# Autodesk Inventor assembly: Hand Assembly V1
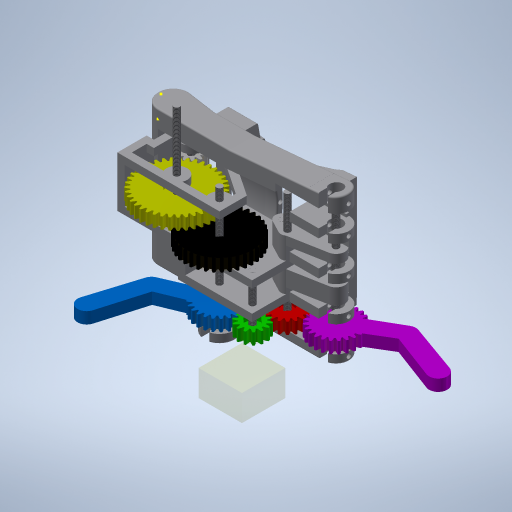
[picture p0: Inventor's stored thumbnail of the model, 512x512]
Saved by Autodesk Inventor 2023 (Build 270158000, 158)
## iProperties
Created: 2016-09-27
Part Number: Hand Assembly V1
Document SubType Name: Assembly
Designer: cmcdona
Author: cmcdona
## Documents named in this file (22)
- C:\Users\manny\OneDrive\Desktop\1C03 Stuff\Hand Assembly\Hand Assembly V1.iam
- C:\Users\manny\OneDrive\Desktop\1C03 Stuff\Hand Assembly\Hand - Frame.ipt
- C:\Users\manny\OneDrive\Desktop\1C03 Stuff\Hand Assembly\Hand - Digit 4.ipt
- C:\Users\manny\OneDrive\Desktop\1C03 Stuff\Hand Assembly\Hand - Digit 0-1.ipt
- C:\Users\manny\OneDrive\Desktop\1C03 Stuff\Hand Assembly\Hand - Distal Bridge.ipt
- C:\Users\manny\OneDrive\Desktop\1C03 Stuff\Hand Assembly\Hand - Digit 2-3.ipt
- C:\Users\manny\OneDrive\Desktop\1C03 Stuff\Hand Assembly\Hand - Proximal Bridge.ipt
- C:\Users\manny\OneDrive\Desktop\1C03 Stuff\Hand Assembly\Hand - Functional Workspace.ipt
- C:\Users\manny\OneDrive\Desktop\1C03 Stuff\Hand Assembly\Input Motor.ipt
- C:\Users\manny\OneDrive\Desktop\1C03 Stuff\Hand Assembly\Spur Gear11.ipt
- C:\Users\manny\OneDrive\Desktop\1C03 Stuff\Hand Assembly\Spur Gear22.ipt
- C:\Users\manny\OneDrive\Desktop\1C03 Stuff\Hand Assembly\temp back plate.ipt
- C:\Users\manny\OneDrive\Desktop\1C03 Stuff\Hand Assembly\Spur Gear12.ipt
- C:\Users\manny\OneDrive\Desktop\1C03 Stuff\Hand Assembly\Spur Gear23.ipt
- C:\Users\manny\OneDrive\Desktop\1C03 Stuff\Hand Assembly\Spur Gear21.ipt
- C:\Users\manny\OneDrive\Desktop\1C03 Stuff\Hand Assembly\FrameAssembly(Printing).iam
- C:\Users\manny\OneDrive\Desktop\1C03 Stuff\Hand Assembly\Spur Gear6.ipt
- C:\Users\manny\OneDrive\Desktop\1C03 Stuff\Hand Assembly\Spur Gear7.ipt
- C:\Users\manny\OneDrive\Desktop\1C03 Stuff\Hand Assembly\Threaded Rod.ipt
- C:\Users\manny\OneDrive\Desktop\1C03 Stuff\Hand Assembly\Threaded Rod 30mm.ipt
- C:\Users\manny\OneDrive\Desktop\1C03 Stuff\Hand Assembly\Threaded Rod38 mm.ipt
- C:\Users\manny\OneDrive\Desktop\1C03 Stuff\Hand Assembly\Threaded Rod 46mm.ipt
## Components (27 placed, 16 different names)
1. Hand - Frame:1 — Flush:1, Flush:2, Mate:1, Mate:2, Flush:3, Mate:3, Mate:16, Mate:17, Mate:18, Mate:33, Mate:34, Mate:53, Mate:66
2. Hand - Digit 4:1 — Flush:1, Flush:2, Mate:1, Mate:4, Mate:5
3. Hand - Digit 0-1:1 — Mate:2, Flush:3, Mate:3, Mate:6, Mate:19, Mate:20, Mate:21, Mate:31, Mate:58, Mate:59, Mate:63, Flush:21
4. Hand - Distal Bridge:1 — Mate:4, Mate:5, Mate:6, Mate:7, Mate:8, Mate:9, Mate:10, Mate:11, Mate:12, Mate:13, Mate:14, Mate:15
5. Hand - Digit 2-3:1 — Mate:7, Mate:8, Mate:9
6. Hand - Digit 2-3:2 — Mate:10, Mate:11, Mate:12
7. Hand - Digit 2-3:3 — Mate:13, Mate:14, Mate:15
8. Hand - Proximal Bridge:1 — Mate:16, Mate:17, Mate:18
9. Hand - Functional Workspace:1 — Mate:19, Mate:20, Mate:21
10. Input Motor:1 — Mate:24, Mate:25, Mate:32, Mate:33, Mate:34, Mate:53, Mate:54, Mate:65
11. Spur Gear1:1 — Mate:24, Flush:11, Mate:54, Tangent:3, Rotation:4
12. Spur Gear2:1 — Mate:27, Flush:11, Mate:64, Tangent:3, Mate:71, Mate:72, Rotation:4
13. Spur Gear1:2 — Mate:27, Mate:64, Flush:20, Tangent:2, Mate:71, Rotation:5
14. Spur Gear2:2 — Mate:31, Flush:20, Tangent:2, Mate:70, Rotation:5
15. Spur Gear2:3 — Mate:58, Mate:63, Flush:22, Rotation:1, Mate:70, Flush:27, Mate:76
16. Spur Gear2:4 — Mate:59, Mate:69, Rotation:3, Flush:24, Mate:73
17. Spur Gear1:3 — Mate:67, Flush:22, Flush:23, Rotation:1, Rotation:2, Mate:79, Flush:30
18. Spur Gear2:5 — Mate:68, Flush:23, Rotation:2, Rotation:3, Flush:25, Mate:74
19. FrameAssembly(Printing):1 [sub-assembly] — Mate:65, Flush:21, Mate:66, Mate:67, Mate:68, Mate:69, Mate:72, Flush:28, Mate:77, Flush:29, Mate:78, Mate:80, Flush:31
20. temp back plate:1 — Mate:25, Mate:32
21. Threaded Rod:1 — Flush:24, Mate:73
22. Threaded Rod:2 — Flush:25, Mate:74
23. Threaded Rod:4 — Flush:27, Mate:76
24. Threaded Rod:5 — Flush:28, Mate:77
25. Threaded Rod 30mm:1 — Flush:29, Mate:78
26. Threaded Rod38 mm:1 — Mate:79, Flush:30
27. Threaded Rod 46mm:1 — Mate:80, Flush:31
## Relationships (71: Mate 49, Flush 15, RelateRotation 5, Tangent 2)
- Flush:1: Hand - Frame:1 ↔ Hand - Digit 4:1
- Flush:2: Hand - Frame:1 ↔ Hand - Digit 4:1
- Mate:1: Hand - Frame:1 ↔ Hand - Digit 4:1
- Mate:2: Hand - Frame:1 ↔ Hand - Digit 0-1:1
- Flush:3: Hand - Frame:1 ↔ Hand - Digit 0-1:1
- Mate:3: Hand - Frame:1 ↔ Hand - Digit 0-1:1
- Mate:4: Hand - Digit 4:1 ↔ Hand - Distal Bridge:1
- Mate:5: Hand - Digit 4:1 ↔ Hand - Distal Bridge:1
- Mate:6: Hand - Digit 0-1:1 ↔ Hand - Distal Bridge:1
- Mate:7: Hand - Distal Bridge:1 ↔ Hand - Digit 2-3:1
- Mate:8: Hand - Distal Bridge:1 ↔ Hand - Digit 2-3:1
- Mate:9: Hand - Distal Bridge:1 ↔ Hand - Digit 2-3:1
- Mate:10: Hand - Distal Bridge:1 ↔ Hand - Digit 2-3:2
- Mate:11: Hand - Distal Bridge:1 ↔ Hand - Digit 2-3:2
- Mate:12: Hand - Distal Bridge:1 ↔ Hand - Digit 2-3:2
- Mate:13: Hand - Distal Bridge:1 ↔ Hand - Digit 2-3:3
- Mate:14: Hand - Distal Bridge:1 ↔ Hand - Digit 2-3:3
- Mate:15: Hand - Distal Bridge:1 ↔ Hand - Digit 2-3:3
- Mate:16: Hand - Frame:1 ↔ Hand - Proximal Bridge:1
- Mate:17: Hand - Frame:1 ↔ Hand - Proximal Bridge:1
- Mate:18: Hand - Frame:1 ↔ Hand - Proximal Bridge:1
- Mate:19: Hand - Digit 0-1:1 ↔ Hand - Functional Workspace:1
- Mate:20 (41 mm): Hand - Digit 0-1:1 ↔ Hand - Functional Workspace:1
- Mate:21 (33 mm): Hand - Digit 0-1:1 ↔ Hand - Functional Workspace:1
- Mate:24: Input Motor:1 ↔ Spur Gear1:1
- Mate:25: Input Motor:1 ↔ temp back plate:1
- Mate:27: Spur Gear2:1 ↔ Spur Gear1:2
- Mate:31: Hand - Digit 0-1:1 ↔ Spur Gear2:2
- Mate:32: Input Motor:1 ↔ temp back plate:1
- Mate:33: Hand - Frame:1 ↔ Input Motor:1
- Mate:34: Hand - Frame:1 ↔ Input Motor:1
- Mate:53 (1 mm): Hand - Frame:1 ↔ Input Motor:1
- Flush:11: Spur Gear1:1 ↔ Spur Gear2:1
- Mate:54 (3 mm): Input Motor:1 ↔ Spur Gear1:1
- Mate:58: Hand - Digit 0-1:1 ↔ Spur Gear2:3
- Mate:59 (5 mm): Hand - Digit 0-1:1 ↔ Spur Gear2:4
- Mate:63 (5 mm): Hand - Digit 0-1:1 ↔ Spur Gear2:3
- Mate:64: Spur Gear2:1 ↔ Spur Gear1:2
- Flush:20: Spur Gear1:2 ↔ Spur Gear2:2
- Mate:65: Input Motor:1 ↔ FrameAssembly(Printing):1
- Flush:21: Hand - Digit 0-1:1 ↔ FrameAssembly(Printing):1
- Mate:66 (2 mm): Hand - Frame:1 ↔ FrameAssembly(Printing):1
- Mate:67: Spur Gear1:3 ↔ FrameAssembly(Printing):1
- Mate:68: Spur Gear2:5 ↔ FrameAssembly(Printing):1
- Flush:22: Spur Gear2:3 ↔ Spur Gear1:3
- Flush:23: Spur Gear1:3 ↔ Spur Gear2:5
- Mate:69: Spur Gear2:4 ↔ FrameAssembly(Printing):1
- Tangent:2: Spur Gear1:2 ↔ Spur Gear2:2
- Tangent:3: Spur Gear1:1 ↔ Spur Gear2:1
- Rotation:1 [RelateRotation] (1.714 ul): Spur Gear2:3 ↔ Spur Gear1:3
- Rotation:2 [RelateRotation] (0.7 ul): Spur Gear1:3 ↔ Spur Gear2:5
- Rotation:3 [RelateRotation] (0.833 ul): Spur Gear2:4 ↔ Spur Gear2:5
- Mate:70: Spur Gear2:2 ↔ Spur Gear2:3
- Mate:71: Spur Gear2:1 ↔ Spur Gear1:2
- Mate:72: Spur Gear2:1 ↔ FrameAssembly(Printing):1
- Rotation:4 [RelateRotation] (0.308 ul): Spur Gear1:1 ↔ Spur Gear2:1
- Rotation:5 [RelateRotation] (0.333 ul): Spur Gear1:2 ↔ Spur Gear2:2
- Flush:24: Spur Gear2:4 ↔ Threaded Rod:1
- Mate:73: Spur Gear2:4 ↔ Threaded Rod:1
- Flush:25: Spur Gear2:5 ↔ Threaded Rod:2
- Mate:74: Spur Gear2:5 ↔ Threaded Rod:2
- Flush:27: Spur Gear2:3 ↔ Threaded Rod:4
- Mate:76: Spur Gear2:3 ↔ Threaded Rod:4
- Flush:28: FrameAssembly(Printing):1 ↔ Threaded Rod:5
- Mate:77: FrameAssembly(Printing):1 ↔ Threaded Rod:5
- Flush:29 (5 mm): FrameAssembly(Printing):1 ↔ Threaded Rod 30mm:1
- Mate:78: FrameAssembly(Printing):1 ↔ Threaded Rod 30mm:1
- Mate:79: Spur Gear1:3 ↔ Threaded Rod38 mm:1
- Flush:30: Spur Gear1:3 ↔ Threaded Rod38 mm:1
- Mate:80: FrameAssembly(Printing):1 ↔ Threaded Rod 46mm:1
- Flush:31: FrameAssembly(Printing):1 ↔ Threaded Rod 46mm:1
